# Autodesk Inventor assembly: DriveWheelAssembly
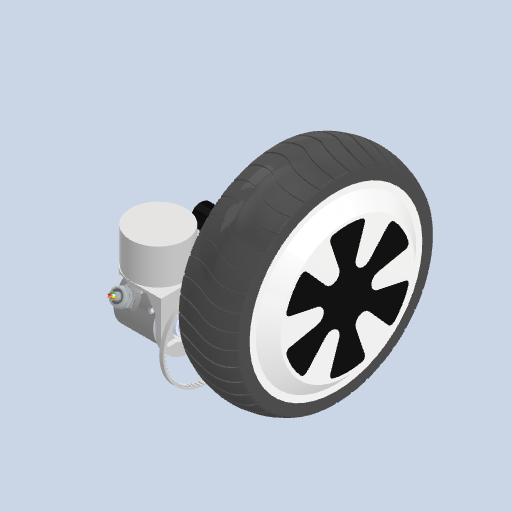
[picture p0: Inventor's stored thumbnail of the model, 512x512]
Saved by Autodesk Inventor 2023 (Build 270158000, 158)
## iProperties
Created: 2022-12-26
Part Number: DriveWheelAssembly
Document SubType Name: Assembly
Designer: haash
Author: haash
## Documents named in this file (8)
- C:\Users\haash\OneDrive\Documents\Projects\Hoverboard-Robot\DriveWheelAssembly.iam
- C:\Users\haash\OneDrive\Documents\Projects\Hoverboard-Robot\Hoverboard-Wheel\Motor, BLDC, Hoverboard Wheel, 6.5in.ipt
- C:\Users\haash\OneDrive\Documents\Projects\Hoverboard-Robot\Hoverboard Frame.ipt
- C:\Users\haash\OneDrive\Documents\Projects\Hoverboard-Robot\EncoderTimingBelt.ipt
- C:\Users\haash\OneDrive\Documents\Projects\Hoverboard-Robot\EncoderPully.ipt
- C:\Users\haash\OneDrive\Documents\Projects\Hoverboard-Robot\WheelPully.ipt
- C:\Users\haash\OneDrive\Documents\Projects\Hoverboard-Robot\EncoderMount.ipt
- C:\Users\haash\OneDrive\Documents\Projects\Hoverboard-Robot\Encoder\38 mm OD, 6 mm Shaft, Incremental Optical Rotary Encoder.iam
## Components (7 placed, 7 different names)
1. Motor, BLDC, Hoverboard Wheel, 6.5in:1
2. Hoverboard Frame:1
3. EncoderTimingBelt:1
4. EncoderPully:1
5. WheelPully:1
6. EncoderMount:1
7. 38 mm OD, 6 mm Shaft, Incremental Optical Rotary Encoder:1 [sub-assembly]
## Relationships (13: Mate 12, Angle 1)
- [Mate]: Motor, BLDC, Hoverboard Wheel, 6.5in:1 ↔ WheelPully:1
- [Mate]: Motor, BLDC, Hoverboard Wheel, 6.5in:1 ↔ EncoderTimingBelt:1
- [Mate]: Hoverboard Frame:1 ↔ EncoderMount:1
- [Mate]: Hoverboard Frame:1 ↔ EncoderMount:1
- [Mate]: Hoverboard Frame:1 ↔ EncoderMount:1
- [Mate]: EncoderMount:1 ↔ 38 mm OD, 6 mm Shaft, Incremental Optical Rotary Encoder:1
- [Mate]: EncoderMount:1 ↔ 38 mm OD, 6 mm Shaft, Incremental Optical Rotary Encoder:1
- [Mate]: EncoderPully:1 ↔ WheelPully:1
- [Mate]: Motor, BLDC, Hoverboard Wheel, 6.5in:1 ↔ WheelPully:1
- [Angle] (0 deg): EncoderMount:1 ↔ 38 mm OD, 6 mm Shaft, Incremental Optical Rotary Encoder:1
- [Mate]: EncoderPully:1 ↔ 38 mm OD, 6 mm Shaft, Incremental Optical Rotary Encoder:1
- [Mate]: EncoderTimingBelt:1 ↔ EncoderPully:1
- [Mate]: EncoderTimingBelt:1 ↔ WheelPully:1
